# Autodesk Inventor assembly: 2号螺丝+螺帽
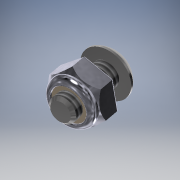
[picture p0: Inventor's stored thumbnail of the model, 180x180]
Saved by Autodesk Inventor 2019.4 (Build 234330000, 330)
## iProperties
Created: 2018-09-03
Part Number: 2号螺丝+螺帽
Material: 常规
Document SubType Name: Assembly
Designer: aresp
Mass: 2.87681 g
Surface Area: 5.14039 cm^2
Volume: 0.40742 cm^3
Density: 7.06104 g/cm^3
Author: aresp
## Documents named in this file (3)
- C:\towerTakeOverCad\ncrCadLib\2号螺丝+螺帽.iam
- C:\towerTakeOverCad\ncrCadLib\螺丝螺帽\Screw 8-32 x 0.375'' - Black.ipt
- C:\towerTakeOverCad\ncrCadLib\螺丝螺帽\Nut 8-32 Nylock.ipt
## Components (2 placed, 2 different names)
1. Screw 8-32 x 0.375'' - Black:1 — 配合:2
2. Nut 8-32 Nylock:1 — 配合:2
## Relationships (2: Mate 2)
- [Mate]: Screw 8-32 x 0.375'' - Black:1 ↔ Nut 8-32 Nylock:1
- 配合:2 [Mate] (3.15 mm): Screw 8-32 x 0.375'' - Black:1 ↔ Nut 8-32 Nylock:1
